# Autodesk Inventor assembly: wheel_axle_MIR
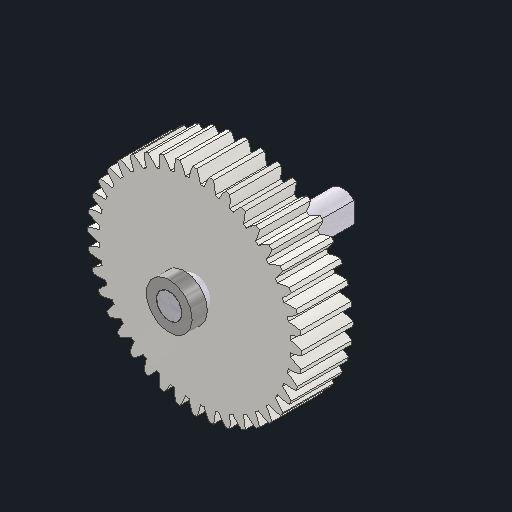
[picture p0: Inventor's stored thumbnail of the model, 512x512]
Saved by Autodesk Inventor 2023 (Build 270158000, 158)
## iProperties
Created: 2024-04-09
Part Number: wheel_axle_MIR
Document SubType Name: Assembly
Designer: szymo
Mass: 22 g
Surface Area: 63.6068 cm^2
Volume: 13.7138 cm^3
TOTAL MASS: 0.0
Author: szymo
## Documents named in this file (6)
- D:\roboilo\robots\codename wafel - australia\3d_parts\rev4\wheel_axle_MIR.iam
- D:\roboilo\robots\codename wafel - australia\3d_parts\rev4\wal_kola_MIR.ipt
- D:\roboilo\robots\codename wafel - australia\3d_parts\rev4\MegaSumo kola zebate 38.ipt
- D:\roboilo\robots\codename wafel - australia\3d_parts\rev4\small_bearing_MIR.ipt
- D:\roboilo\robots\codename wafel - australia\3d_parts\rev4\big_bearing_MIR.ipt
- D:\roboilo\robots\codename wafel - australia\3d_parts\rev4\Design Accelerator\big_gear3_MIR.iam
## Components (5 placed, 5 different names)
1. wal_kola_MIR:1 — Mate:4, Mate:3, Mate:6, Mate:5, Angle:1
2. MegaSumo kola zebate 38:1
3. small_bearing_MIR:1 — Mate:4, Mate:3
4. big_bearing_MIR:1 — Mate:6, Mate:5
5. big_gear3_MIR:1 [sub-assembly] — Angle:1
## Relationships (5: Mate 4, Angle 1)
- Mate:4: wal_kola_MIR:1 ↔ small_bearing_MIR:1
- Mate:3: wal_kola_MIR:1 ↔ small_bearing_MIR:1
- Mate:6: wal_kola_MIR:1 ↔ big_bearing_MIR:1
- Mate:5: wal_kola_MIR:1 ↔ big_bearing_MIR:1
- Angle:1 (0 deg): wal_kola_MIR:1 ↔ big_gear3_MIR:1
